# Autodesk Inventor assembly: x_gantry
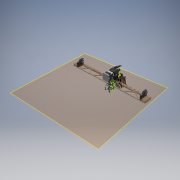
[picture p0: Inventor's stored thumbnail of the model, 180x180]
Saved by Autodesk Inventor 2017 (Build 210142000, 142)
## iProperties
Created: 2016-06-03
Part Number: x_gantry
Document SubType Name: Assembly
Designer: brent
Author: brent
## Documents named in this file (12)
- C:\Users\yibre\OneDrive\personal\printer_mechanical\x_gantry.iam
- C:\Users\yibre\OneDrive\personal\printer_mechanical\xaxis.ipt
- C:\Users\yibre\OneDrive\personal\printer_mechanical\extruder\extruder_175mm.iam
- C:\Users\yibre\OneDrive\personal\printer_mechanical\offtheshelf\mgn9_350mm.ipt
- C:\Users\yibre\OneDrive\personal\printer_mechanical\offtheshelf\mgn9h_carriage.ipt
- C:\Users\yibre\OneDrive\personal\printer_mechanical\geometry.ipt
- C:\Users\yibre\OneDrive\personal\printer_mechanical\offtheshelf\623bearing.ipt
- C:\Users\yibre\OneDrive\personal\printer_mechanical\spacers\idler_flange.ipt
- C:\Users\yibre\OneDrive\personal\printer_mechanical\x_gantry\Design Accelerator\Bolted Connection1.iam
- C:\Users\yibre\OneDrive\personal\printer_mechanical\x_gantry\Design Accelerator\Bolted Connection2.iam
- C:\Users\yibre\OneDrive\personal\printer_mechanical\x_gantry\Design Accelerator\Bolted Connection1_MIR.iam
- C:\Users\yibre\OneDrive\personal\printer_mechanical\x_gantry\Design Accelerator\Bolted Connection2_MIR.iam
## Components (21 placed, 10 different names)
1. xaxis:1 — Mate:1, Mate:2, Mate:3, Mate:9, Mate:10, Mate:11, Mate:12, Mate:13, Mate:14, Flush:1, Flush:2, Mate:22, Mate:31, Mate:34, Mate:35, Mate:36, Mate:37, Mate:38, Mate:39, Mate:40, Mate:41
2. extruder_175mm:1 [sub-assembly] — Mate:6, Mate:7, Mate:8
3. mgn9_350mm:1 — Mate:1, Mate:2, Mate:3, Mate:4, Mate:5
4. mgn9h_carriage:1 — Mate:4, Mate:5, Mate:6, Mate:7, Mate:8
5. mgn9h_carriage:2 — Mate:9, Mate:10, Mate:11
6. mgn9h_carriage:3 — Mate:12, Mate:13, Mate:14
7. geometry:1 — Flush:2, Mate:23, Flush:3, Mate:32, Mate:33
8. 623bearing:1 — Mate:15, Mate:18, Mate:22, Mate:23
9. 623bearing:2 — Mate:15, Mate:18, Mate:19, Mate:21
10. 623bearing:3 — Mate:16, Mate:17, Mate:19, Mate:20
11. 623bearing:4 — Mate:16, Mate:17, Flush:3
12. 623bearing:5 — Mate:24, Mate:25, Mate:28, Mate:31, Mate:32
13. 623bearing:6 — Mate:25, Mate:28, Mate:29, Mate:30
14. 623bearing:7 — Mate:24, Mate:26, Mate:27, Mate:33
15. 623bearing:8 — Mate:26, Mate:27
16. idler_flange:1 — Mate:20, Mate:21
17. idler_flange:2 — Mate:29, Mate:30
18. Bolted Connection:1 [sub-assembly] — Mate:34, Mate:35
19. Bolted Connection:2 [sub-assembly] — Mate:36, Mate:37
20. Bolted Connection1_MIR:1 [sub-assembly] — Mate:38, Mate:40
21. Bolted Connection2_MIR:1 [sub-assembly] — Mate:39, Mate:41
## Relationships (44: Mate 41, Flush 3)
- Mate:1: xaxis:1 ↔ mgn9_350mm:1
- Mate:2: xaxis:1 ↔ mgn9_350mm:1
- Mate:3: xaxis:1 ↔ mgn9_350mm:1
- Mate:4: mgn9_350mm:1 ↔ mgn9h_carriage:1
- Mate:5: mgn9_350mm:1 ↔ mgn9h_carriage:1
- Mate:6: extruder_175mm:1 ↔ mgn9h_carriage:1
- Mate:7: extruder_175mm:1 ↔ mgn9h_carriage:1
- Mate:8: extruder_175mm:1 ↔ mgn9h_carriage:1
- Mate:9: xaxis:1 ↔ mgn9h_carriage:2
- Mate:10: xaxis:1 ↔ mgn9h_carriage:2
- Mate:11: xaxis:1 ↔ mgn9h_carriage:2
- Mate:12: xaxis:1 ↔ mgn9h_carriage:3
- Mate:13: xaxis:1 ↔ mgn9h_carriage:3
- Mate:14: xaxis:1 ↔ mgn9h_carriage:3
- Flush:1 (10 mm): xaxis:1
- Flush:2: xaxis:1 ↔ geometry:1
- Mate:15: 623bearing:1 ↔ 623bearing:2
- Mate:16: 623bearing:3 ↔ 623bearing:4
- Mate:17: 623bearing:3 ↔ 623bearing:4
- Mate:18: 623bearing:1 ↔ 623bearing:2
- Mate:19: 623bearing:2 ↔ 623bearing:3
- Mate:20: 623bearing:3 ↔ idler_flange:1
- Mate:21: 623bearing:2 ↔ idler_flange:1
- Mate:22: xaxis:1 ↔ 623bearing:1
- Mate:23: geometry:1 ↔ 623bearing:1
- Flush:3: geometry:1 ↔ 623bearing:4
- Mate:24: 623bearing:5 ↔ 623bearing:7
- Mate:25: 623bearing:5 ↔ 623bearing:6
- Mate:26: 623bearing:7 ↔ 623bearing:8
- Mate:27: 623bearing:7 ↔ 623bearing:8
- Mate:28: 623bearing:5 ↔ 623bearing:6
- Mate:29: 623bearing:6 ↔ idler_flange:2
- Mate:30: 623bearing:6 ↔ idler_flange:2
- Mate:31: xaxis:1 ↔ 623bearing:5
- Mate:32: geometry:1 ↔ 623bearing:5
- Mate:33: geometry:1 ↔ 623bearing:7
- Mate:34: xaxis:1 ↔ Bolted Connection:1
- Mate:35: xaxis:1 ↔ Bolted Connection:1
- Mate:36: xaxis:1 ↔ Bolted Connection:2
- Mate:37: xaxis:1 ↔ Bolted Connection:2
- Mate:38: xaxis:1 ↔ Bolted Connection1_MIR:1
- Mate:39: xaxis:1 ↔ Bolted Connection2_MIR:1
- Mate:40: xaxis:1 ↔ Bolted Connection1_MIR:1
- Mate:41: xaxis:1 ↔ Bolted Connection2_MIR:1
